# Autodesk Inventor assembly: 42146-06
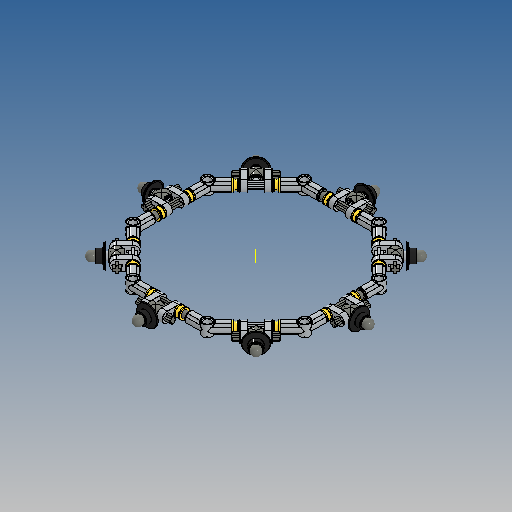
[picture p0: Inventor's stored thumbnail of the model, 512x512]
Saved by Autodesk Inventor 2025 (Build 290162010, 162A)
## iProperties
Created: 2024-11-15
Part Number: 42146-06
Material: Generisch
Document SubType Name: Assembly
Designer: hp.muther
Author: hp.muther
## Documents named in this file (10)
- D:\Inventor\Projekte\Muther\LEGO Technic\LEGO Technik - Raupenkran LR 13000 (42146)\42146-01-06.iam
- D:\Inventor\Projekte\Muther\LEGO Technic\LEGO Pieces\Achsen\32209-DkBluishGray.ipt
- D:\Inventor\Projekte\Muther\LEGO Technic\LEGO Pieces\Achsen\32073-LtBluishGray.ipt
- D:\Inventor\Projekte\Muther\LEGO Technic\LEGO Pieces\Verbindungselemente mit Pin\27940-DkBluishGray.ipt
- D:\Inventor\Projekte\Muther\LEGO Technic\LEGO Pieces\Rund\4265c-Yellow.ipt
- D:\Inventor\Projekte\Muther\LEGO Technic\LEGO Pieces\Lochbalken schmal\41677-LtBluishGray.ipt
- D:\Inventor\Projekte\Muther\LEGO Technic\LEGO Pieces\Pin's\4274-LtBluishGray.ipt
- D:\Inventor\Projekte\Muther\LEGO Technic\LEGO Pieces\Diverses\22484-DkBluishGray.ipt
- D:\Inventor\Projekte\Muther\LEGO Technic\LEGO Pieces\Räder, Raupe\50254-Black.ipt
- D:\Inventor\Projekte\Muther\LEGO Technic\LEGO Pieces\Verbindungselemente\32192-LtBluishGray.ipt
## Components (80 placed, 9 different names)
1. 32192-LtBluishGray:1 — Einfügen:1
2. 32209-DkBluishGray:1 — Einfügen:1, Einfügen:2, Passend:1, Passend:2, Passend:3, Passend:5
3. 32073-LtBluishGray:1 — Einfügen:14, Passend:7, Passend:8, Passend:9, Passend:10, Passend:20
4. 27940-DkBluishGray:1 — Einfügen:4, Einfügen:5, Einfügen:7
5. 4265c-Yellow:1 — Einfügen:2, Passend:1, Einfügen:3
6. 41677-LtBluishGray:1 — Einfügen:3, Passend:2, Einfügen:4
7. 41677-LtBluishGray:2 — Einfügen:5, Einfügen:6
8. 4265c-Yellow:2 — Einfügen:6, Passend:3, Einfügen:8
9. 4274-LtBluishGray:1 — Einfügen:7, Einfügen:16
10. 32192-LtBluishGray:2 — Einfügen:8, Passend:5, Einfügen:14, Einfügen:15
11. 27940-DkBluishGray:2
12. 4265c-Yellow:3 — Einfügen:15, Passend:7
13. 41677-LtBluishGray:3 — Passend:8
14. 41677-LtBluishGray:4 — Passend:9
15. 4265c-Yellow:4 — Passend:10, Einfügen:39
16. 4274-LtBluishGray:2 — Einfügen:17
17. 22484-DkBluishGray:1 — Einfügen:18
18. 22484-DkBluishGray:2 — Einfügen:19
19. 50254-Black:1 — Einfügen:16, Einfügen:18
20. 50254-Black:2 — Einfügen:17, Einfügen:19, Symmetrie:2
21. 32192-LtBluishGray:3 — Einfügen:39, Passend:20
22. 32209-DkBluishGray:2
23. 32073-LtBluishGray:2 — Passend:40
24. 27940-DkBluishGray:3
25. 4265c-Yellow:5
26. 41677-LtBluishGray:5
27. 41677-LtBluishGray:6
28. 4265c-Yellow:6 — Einfügen:28
29. 4274-LtBluishGray:3
30. 22484-DkBluishGray:3
31. 32192-LtBluishGray:4 — Einfügen:28, Einfügen:35
32. 27940-DkBluishGray:4
33. 4265c-Yellow:7 — Einfügen:35
34. 41677-LtBluishGray:7
35. 41677-LtBluishGray:8
36. 4265c-Yellow:8 — Einfügen:79
37. 4274-LtBluishGray:4
38. 22484-DkBluishGray:4
39. 50254-Black:3
40. 50254-Black:4 — Symmetrie:3
41. 32192-LtBluishGray:5 — Einfügen:79, Passend:40
42. 32209-DkBluishGray:3
43. 32073-LtBluishGray:3
44. 27940-DkBluishGray:5
45. 4265c-Yellow:9
46. 41677-LtBluishGray:9
47. 41677-LtBluishGray:10
48. 4265c-Yellow:10
49. 4274-LtBluishGray:5
50. 22484-DkBluishGray:5
51. 32192-LtBluishGray:6
52. 27940-DkBluishGray:6
53. 4265c-Yellow:11
54. 41677-LtBluishGray:11
55. 41677-LtBluishGray:12
56. 4265c-Yellow:12
57. 4274-LtBluishGray:6
58. 22484-DkBluishGray:6
59. 50254-Black:5
60. 50254-Black:6 — Symmetrie:2
61. 32192-LtBluishGray:7
62. 32209-DkBluishGray:4
63. 32073-LtBluishGray:4
64. 27940-DkBluishGray:7
65. 4265c-Yellow:13
66. 41677-LtBluishGray:13
67. 41677-LtBluishGray:14
68. 4265c-Yellow:14
69. 4274-LtBluishGray:7
70. 22484-DkBluishGray:7
71. 32192-LtBluishGray:8
72. 27940-DkBluishGray:8
73. 4265c-Yellow:15
74. 41677-LtBluishGray:15
75. 41677-LtBluishGray:16
76. 4265c-Yellow:16
77. 4274-LtBluishGray:8
78. 22484-DkBluishGray:8
79. 50254-Black:7
80. 50254-Black:8 — Symmetrie:3
## Relationships (122: Insert 79, Mate 41, Symmetry 2)
- Einfügen:1 [Insert]: 32192-LtBluishGray:1 ↔ 32209-DkBluishGray:1
- Einfügen:2 [Insert]: 32209-DkBluishGray:1 ↔ 4265c-Yellow:1
- Passend:1 [Mate]: 32209-DkBluishGray:1 ↔ 4265c-Yellow:1
- Einfügen:3 [Insert]: 4265c-Yellow:1 ↔ 41677-LtBluishGray:1
- Passend:2 [Mate]: 32209-DkBluishGray:1 ↔ 41677-LtBluishGray:1
- Einfügen:4 [Insert]: 27940-DkBluishGray:1 ↔ 41677-LtBluishGray:1
- Einfügen:5 [Insert]: 27940-DkBluishGray:1 ↔ 41677-LtBluishGray:2
- Einfügen:6 [Insert]: 41677-LtBluishGray:2 ↔ 4265c-Yellow:2
- Passend:3 [Mate]: 32209-DkBluishGray:1 ↔ 4265c-Yellow:2
- Einfügen:7 [Insert]: 27940-DkBluishGray:1 ↔ 4274-LtBluishGray:1
- Einfügen:18 [Insert]: 22484-DkBluishGray:1 ↔ 50254-Black:1
- Einfügen:8 [Insert]: 4265c-Yellow:2 ↔ 32192-LtBluishGray:2
- Passend:5 [Mate]: 32209-DkBluishGray:1 ↔ 32192-LtBluishGray:2
- [Insert]: 4265c-Yellow:3 ↔ 41677-LtBluishGray:3
- [Insert]: 27940-DkBluishGray:2 ↔ 41677-LtBluishGray:3
- [Insert]: 27940-DkBluishGray:2 ↔ 41677-LtBluishGray:4
- [Insert]: 41677-LtBluishGray:4 ↔ 4265c-Yellow:4
- [Insert]: 27940-DkBluishGray:2 ↔ 4274-LtBluishGray:2
- [Mate]: 4274-LtBluishGray:2 ↔ 22484-DkBluishGray:2
- Einfügen:14 [Insert] (-8 mm): 32073-LtBluishGray:1 ↔ 32192-LtBluishGray:2
- Einfügen:15 [Insert]: 32192-LtBluishGray:2 ↔ 4265c-Yellow:3
- Passend:7 [Mate]: 32073-LtBluishGray:1 ↔ 4265c-Yellow:3
- Passend:8 [Mate]: 32073-LtBluishGray:1 ↔ 41677-LtBluishGray:3
- Passend:9 [Mate]: 32073-LtBluishGray:1 ↔ 41677-LtBluishGray:4
- Passend:10 [Mate]: 32073-LtBluishGray:1 ↔ 4265c-Yellow:4
- Einfügen:16 [Insert]: 4274-LtBluishGray:1 ↔ 50254-Black:1
- Einfügen:17 [Insert]: 4274-LtBluishGray:2 ↔ 50254-Black:2
- Einfügen:19 [Insert]: 22484-DkBluishGray:2 ↔ 50254-Black:2
- [Insert]: 32192-LtBluishGray:3 ↔ 32209-DkBluishGray:2
- [Insert]: 32209-DkBluishGray:2 ↔ 4265c-Yellow:5
- [Mate]: 32209-DkBluishGray:2 ↔ 4265c-Yellow:5
- [Insert]: 4265c-Yellow:5 ↔ 41677-LtBluishGray:5
- [Mate]: 32209-DkBluishGray:2 ↔ 41677-LtBluishGray:5
- [Insert]: 27940-DkBluishGray:3 ↔ 41677-LtBluishGray:5
- [Insert]: 27940-DkBluishGray:3 ↔ 41677-LtBluishGray:6
- [Insert]: 41677-LtBluishGray:6 ↔ 4265c-Yellow:6
- [Mate]: 32209-DkBluishGray:2 ↔ 4265c-Yellow:6
- [Insert]: 27940-DkBluishGray:3 ↔ 4274-LtBluishGray:3
- [Insert]: 22484-DkBluishGray:3 ↔ 50254-Black:3
- Einfügen:28 [Insert]: 4265c-Yellow:6 ↔ 32192-LtBluishGray:4
- [Mate]: 32209-DkBluishGray:2 ↔ 32192-LtBluishGray:4
- [Insert]: 4265c-Yellow:7 ↔ 41677-LtBluishGray:7
- [Insert]: 27940-DkBluishGray:4 ↔ 41677-LtBluishGray:7
- [Insert]: 27940-DkBluishGray:4 ↔ 41677-LtBluishGray:8
- [Insert]: 41677-LtBluishGray:8 ↔ 4265c-Yellow:8
- [Insert]: 27940-DkBluishGray:4 ↔ 4274-LtBluishGray:4
- [Mate]: 4274-LtBluishGray:4 ↔ 22484-DkBluishGray:4
- [Insert] (-8 mm): 32073-LtBluishGray:2 ↔ 32192-LtBluishGray:4
- Einfügen:35 [Insert]: 32192-LtBluishGray:4 ↔ 4265c-Yellow:7
- [Mate]: 32073-LtBluishGray:2 ↔ 4265c-Yellow:7
- [Mate]: 32073-LtBluishGray:2 ↔ 41677-LtBluishGray:7
- [Mate]: 32073-LtBluishGray:2 ↔ 41677-LtBluishGray:8
- [Mate]: 32073-LtBluishGray:2 ↔ 4265c-Yellow:8
- [Insert]: 4274-LtBluishGray:3 ↔ 50254-Black:3
- [Insert]: 4274-LtBluishGray:4 ↔ 50254-Black:4
- [Insert]: 22484-DkBluishGray:4 ↔ 50254-Black:4
- Einfügen:39 [Insert]: 4265c-Yellow:4 ↔ 32192-LtBluishGray:3
- Passend:20 [Mate]: 32073-LtBluishGray:1 ↔ 32192-LtBluishGray:3
- [Insert]: 32192-LtBluishGray:5 ↔ 32209-DkBluishGray:3
- [Insert]: 32209-DkBluishGray:3 ↔ 4265c-Yellow:9
- [Mate]: 32209-DkBluishGray:3 ↔ 4265c-Yellow:9
- [Insert]: 4265c-Yellow:9 ↔ 41677-LtBluishGray:9
- [Mate]: 32209-DkBluishGray:3 ↔ 41677-LtBluishGray:9
- [Insert]: 27940-DkBluishGray:5 ↔ 41677-LtBluishGray:9
- [Insert]: 27940-DkBluishGray:5 ↔ 41677-LtBluishGray:10
- [Insert]: 41677-LtBluishGray:10 ↔ 4265c-Yellow:10
- [Mate]: 32209-DkBluishGray:3 ↔ 4265c-Yellow:10
- [Insert]: 27940-DkBluishGray:5 ↔ 4274-LtBluishGray:5
- [Insert]: 22484-DkBluishGray:5 ↔ 50254-Black:5
- [Insert]: 4265c-Yellow:10 ↔ 32192-LtBluishGray:6
- [Mate]: 32209-DkBluishGray:3 ↔ 32192-LtBluishGray:6
- [Insert]: 4265c-Yellow:11 ↔ 41677-LtBluishGray:11
- [Insert]: 27940-DkBluishGray:6 ↔ 41677-LtBluishGray:11
- [Insert]: 27940-DkBluishGray:6 ↔ 41677-LtBluishGray:12
- [Insert]: 41677-LtBluishGray:12 ↔ 4265c-Yellow:12
- [Insert]: 27940-DkBluishGray:6 ↔ 4274-LtBluishGray:6
- [Mate]: 4274-LtBluishGray:6 ↔ 22484-DkBluishGray:6
- [Insert] (-8 mm): 32073-LtBluishGray:3 ↔ 32192-LtBluishGray:6
- [Insert]: 32192-LtBluishGray:6 ↔ 4265c-Yellow:11
- [Mate]: 32073-LtBluishGray:3 ↔ 4265c-Yellow:11
- [Mate]: 32073-LtBluishGray:3 ↔ 41677-LtBluishGray:11
- [Mate]: 32073-LtBluishGray:3 ↔ 41677-LtBluishGray:12
- [Mate]: 32073-LtBluishGray:3 ↔ 4265c-Yellow:12
- [Insert]: 4274-LtBluishGray:5 ↔ 50254-Black:5
- [Insert]: 4274-LtBluishGray:6 ↔ 50254-Black:6
- [Insert]: 22484-DkBluishGray:6 ↔ 50254-Black:6
- [Insert]: 32192-LtBluishGray:7 ↔ 32209-DkBluishGray:4
- [Insert]: 32209-DkBluishGray:4 ↔ 4265c-Yellow:13
- [Mate]: 32209-DkBluishGray:4 ↔ 4265c-Yellow:13
- [Insert]: 4265c-Yellow:13 ↔ 41677-LtBluishGray:13
- [Mate]: 32209-DkBluishGray:4 ↔ 41677-LtBluishGray:13
- [Insert]: 27940-DkBluishGray:7 ↔ 41677-LtBluishGray:13
- [Insert]: 27940-DkBluishGray:7 ↔ 41677-LtBluishGray:14
- [Insert]: 41677-LtBluishGray:14 ↔ 4265c-Yellow:14
- [Mate]: 32209-DkBluishGray:4 ↔ 4265c-Yellow:14
- [Insert]: 27940-DkBluishGray:7 ↔ 4274-LtBluishGray:7
- [Insert]: 22484-DkBluishGray:7 ↔ 50254-Black:7
- [Insert]: 4265c-Yellow:14 ↔ 32192-LtBluishGray:8
- [Mate]: 32209-DkBluishGray:4 ↔ 32192-LtBluishGray:8
- [Insert]: 4265c-Yellow:15 ↔ 41677-LtBluishGray:15
- [Insert]: 27940-DkBluishGray:8 ↔ 41677-LtBluishGray:15
- [Insert]: 27940-DkBluishGray:8 ↔ 41677-LtBluishGray:16
- [Insert]: 41677-LtBluishGray:16 ↔ 4265c-Yellow:16
- [Insert]: 27940-DkBluishGray:8 ↔ 4274-LtBluishGray:8
- [Mate]: 4274-LtBluishGray:8 ↔ 22484-DkBluishGray:8
- [Insert] (-8 mm): 32073-LtBluishGray:4 ↔ 32192-LtBluishGray:8
- [Insert]: 32192-LtBluishGray:8 ↔ 4265c-Yellow:15
- [Mate]: 32073-LtBluishGray:4 ↔ 4265c-Yellow:15
- [Mate]: 32073-LtBluishGray:4 ↔ 41677-LtBluishGray:15
- [Mate]: 32073-LtBluishGray:4 ↔ 41677-LtBluishGray:16
- [Mate]: 32073-LtBluishGray:4 ↔ 4265c-Yellow:16
- [Insert]: 4274-LtBluishGray:7 ↔ 50254-Black:7
- [Insert]: 4274-LtBluishGray:8 ↔ 50254-Black:8
- [Insert]: 22484-DkBluishGray:8 ↔ 50254-Black:8
- [Insert]: 4265c-Yellow:12 ↔ 32192-LtBluishGray:7
- [Mate]: 32073-LtBluishGray:3 ↔ 32192-LtBluishGray:7
- Einfügen:79 [Insert]: 4265c-Yellow:8 ↔ 32192-LtBluishGray:5
- Passend:40 [Mate]: 32073-LtBluishGray:2 ↔ 32192-LtBluishGray:5
- Passend:41 [Mate]
- Passend:42 [Mate]
- Symmetrie:2: 50254-Black:2 ↔ 50254-Black:6
- Symmetrie:3: 50254-Black:4 ↔ 50254-Black:8
## Named parameters: d13_d9 = 0 mm, d14_d10 = 0 mm, d15_d3 = 0 mm, d16_d5 = 0 mm, d17_d6 = 0 mm, d18_d7 = 0 mm, d28_d25 = 0 mm, d29_d26 = 0 mm, d30_d27 = 0 mm, d31_d0 = 0 mm, d32_d1 = 0 mm, d33_d2 = 0 mm, d34_d3 = 0 mm, d35_d4 = 0 mm, d36_d5 = 0 mm, d37_d6 = 0 mm, d38_d7 = 0 mm, d39_d8 = 0 mm, d40_d9 = 0 mm, d41_d10 = 0 mm, d42_d11 = 0 mm, d43_d12 = 0 mm, d44_d13_d9 = 0 mm, d45_d14_d10 = 0 mm, d46_d15_d3 = 0 mm, d47_d16_d5 = 0 mm, d48_d17_d6 = 0 mm, d49_d18_d7 = 0 mm, d50_d19 = -8 mm, d51_d20 = 0 mm, d52_d21 = 0 mm, d53_d22 = 0 mm, d54_d23 = 0 mm, d55_d24 = 0 mm, d58_d56 = 0 mm, d59_d57 = 0 mm, d60_d25 = 0 mm, d61_d26 = 0 mm, d62_d27 = 0 mm, d63_d28_d25 = 0 mm, d64_d29_d26 = 0 mm, d65_d30_d27 = 0 mm, d66_d31_d0 = 0 mm, d67_d32_d1 = 0 mm, d68_d33_d2 = 0 mm, d69_d34_d3 = 0 mm, d70_d35_d4 = 0 mm, d71_d36_d5 = 0 mm, d72_d37_d6 = 0 mm, d73_d38_d7 = 0 mm, d74_d39_d8 = 0 mm, d75_d40_d9 = 0 mm, d76_d41_d10 = 0 mm, d77_d42_d11 = 0 mm, d78_d43_d12 = 0 mm, d79_d44_d13_d9 = 0 mm, d80_d45_d14_d10 = 0 mm, d81_d46_d15_d3 = 0 mm, d82_d47_d16_d5 = 0 mm, d83_d48_d17_d6 = 0 mm, d84_d49_d18_d7 = 0 mm, d85_d50_d19 = -8 mm, d86_d51_d20 = 0 mm, d87_d52_d21 = 0 mm, d88_d53_d22 = 0 mm, d89_d54_d23 = 0 mm, d90_d55_d24 = 0 mm, d91_d0 = 0 mm, d92_d1 = 0 mm, d93_d2 = 0 mm, d94_d3 = 0 mm, d95_d4 = 0 mm, d96_d5 = 0 mm, d97_d6 = 0 mm, d98_d7 = 0 mm, d99_d8 = 0 mm, d100_d9 = 0 mm, d101_d10 = 0 mm, d102_d11 = 0 mm, d103_d12 = 0 mm, d104_d13_d9 = 0 mm, d105_d14_d10 = 0 mm, d106_d15_d3 = 0 mm, d107_d16_d5 = 0 mm, d108_d17_d6 = 0 mm, d109_d18_d7 = 0 mm, d110_d19 = -8 mm, d111_d20 = 0 mm, d112_d21 = 0 mm, d113_d22 = 0 mm, d114_d23 = 0 mm, d115_d24 = 0 mm
